# Autodesk Inventor assembly: TELJES9
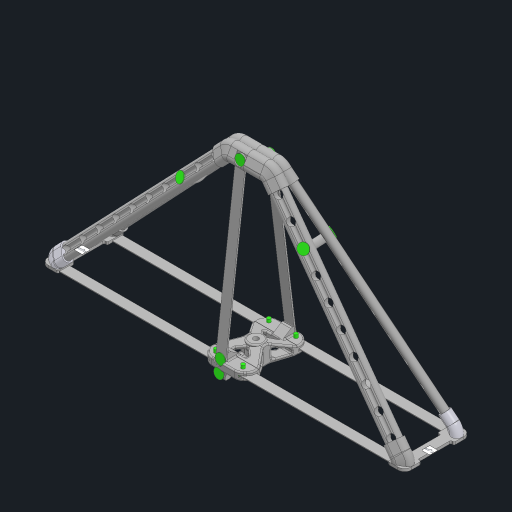
[picture p0: Inventor's stored thumbnail of the model, 512x512]
Saved by Autodesk Inventor 2023 (Build 270158000, 158)
## iProperties
Created: 2022-11-18
Part Number: TELJES9
Document SubType Name: Assembly
Designer: gd1
Author: gd1
## Documents named in this file (15)
- C:\Users\gd1\3D Objects\3D nagyteherbírású híd\Híd\H-d\TELJES9.iam
- C:\Users\gd1\3D Objects\3D nagyteherbírású híd\Híd\H-d\teljes8.iam
- C:\Users\gd1\3D Objects\3D nagyteherbírású híd\Híd\H-d\teljes7.iam
- C:\Users\gd1\3D Objects\3D nagyteherbírású híd\Híd\H-d\TELJES9\AIP\FEA\e5pggsx34.fins
- C:\Users\gd1\3D Objects\3D nagyteherbírású híd\Híd\H-d\TELJES9\AIP\FEA\e5pggsx34.fsat
- C:\Users\gd1\3D Objects\3D nagyteherbírású híd\Híd\H-d\TELJES9\AIP\FEA\e5pggsx34.ftes
- C:\Users\gd1\3D Objects\3D nagyteherbírású híd\Híd\H-d\TELJES9\AIP\FEA\e5pggsx34.fwiz
- C:\Users\gd1\3D Objects\3D nagyteherbírású híd\Híd\H-d\TELJES9\AIP\FEA\e5pggsxq8.fmsh
- C:\Users\gd1\3D Objects\3D nagyteherbírású híd\Híd\H-d\TELJES9\AIP\FEA\e5pggsxq9.fres
- C:\Users\gd1\3D Objects\3D nagyteherbírású híd\Híd\H-d\TELJES9\AIP\FEA\e5u3xwsao.fins
- C:\Users\gd1\3D Objects\3D nagyteherbírású híd\Híd\H-d\TELJES9\AIP\FEA\e5u3xwsao.fsat
- C:\Users\gd1\3D Objects\3D nagyteherbírású híd\Híd\H-d\TELJES9\AIP\FEA\e5u3xwsao.ftes
- C:\Users\gd1\3D Objects\3D nagyteherbírású híd\Híd\H-d\TELJES9\AIP\FEA\e5u3xwsao.fwiz
- C:\Users\gd1\3D Objects\3D nagyteherbírású híd\Híd\H-d\TELJES9\AIP\FEA\e5u3xwuu8.fmsh
- C:\Users\gd1\3D Objects\3D nagyteherbírású híd\Híd\H-d\TELJES9\AIP\FEA\e5u3xwuu9.fres
## Components (2 placed, 2 different names)
1. teljes8:1 [sub-assembly] — Rigid:1
2. teljes7:1 [sub-assembly] — Rigid:1
## Relationships (1: WeldJoint 1)
- Rigid:1 [WeldJoint]: teljes8:1 ↔ teljes7:1
## Named parameters: sa_0 = 500000, sa_1 = 500000
note: some values were not read from the file. Shown as the stored number, unit unknown: "sa_0", "sa_1".
